# Autodesk Inventor assembly: Template A-I
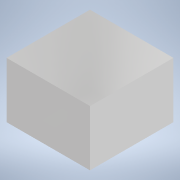
[picture p0: Inventor's stored thumbnail of the model, 180x180]
Saved by Autodesk Inventor 2022 (Build 260153000, 153)
## iProperties
Created: 2022-03-02
Part Number: Template A-I
Document SubType Name: Assembly
Designer: Nathan Griffith
Author: Nathan Griffith
## Documents named in this file (12)
- C:\Users\Nathan Griffith\Documents\Inventor\Eric's Keyboard\Template A-I.iam
- C:\Users\Nathan Griffith\Documents\Inventor\Eric's Keyboard\Block.ipt
- C:\Users\Nathan Griffith\Documents\Inventor\Eric's Keyboard\Keycap a-z\KeycapA.ipt
- C:\Users\Nathan Griffith\Documents\Inventor\Eric's Keyboard\Keycap a-z\KeycapB.ipt
- C:\Users\Nathan Griffith\Documents\Inventor\Eric's Keyboard\Keycap a-z\KeycapC.ipt
- C:\Users\Nathan Griffith\Documents\Inventor\Eric's Keyboard\Keycap a-z\KeycapD.ipt
- C:\Users\Nathan Griffith\Documents\Inventor\Eric's Keyboard\Keycap a-z\KeycapE.ipt
- C:\Users\Nathan Griffith\Documents\Inventor\Eric's Keyboard\Keycap a-z\KeycapF.ipt
- C:\Users\Nathan Griffith\Documents\Inventor\Eric's Keyboard\Keycap a-z\KeycapG.ipt
- C:\Users\Nathan Griffith\Documents\Inventor\Eric's Keyboard\Keycap a-z\KeycapH.ipt
- C:\Users\Nathan Griffith\Documents\Inventor\Eric's Keyboard\Keycap a-z\KeycapI.ipt
- C:\Users\Nathan Griffith\Documents\Inventor\Eric's Keyboard\Holder.iam
## Components (11 placed, 11 different names)
1. Block:1 — Mate:1, Mate:2, Mate:3, Mate:4, Mate:5, Mate:6, Mate:7, Mate:8, Mate:9, Mate:10, Mate:11, Mate:12, Mate:13, Mate:14, Mate:15, Mate:16, Mate:17, Mate:18
2. KeycapA:1 — Mate:1, Mate:2
3. KeycapB:1 — Mate:3, Mate:4
4. KeycapC:1 — Mate:5, Mate:6
5. KeycapD:1 — Mate:7, Mate:8
6. KeycapE:1 — Mate:9, Mate:10
7. KeycapF:1 — Mate:11, Mate:12
8. KeycapG:1 — Mate:13, Mate:14
9. KeycapH:1 — Mate:15, Mate:16
10. KeycapI:1 — Mate:17, Mate:18
11. Holder:1 [sub-assembly]
## Relationships (18: Mate 18)
- Mate:1: Block:1 ↔ KeycapA:1
- Mate:2: Block:1 ↔ KeycapA:1
- Mate:3: Block:1 ↔ KeycapB:1
- Mate:4: Block:1 ↔ KeycapB:1
- Mate:5: Block:1 ↔ KeycapC:1
- Mate:6: Block:1 ↔ KeycapC:1
- Mate:7: Block:1 ↔ KeycapD:1
- Mate:8: Block:1 ↔ KeycapD:1
- Mate:9: Block:1 ↔ KeycapE:1
- Mate:10: Block:1 ↔ KeycapE:1
- Mate:11: Block:1 ↔ KeycapF:1
- Mate:12: Block:1 ↔ KeycapF:1
- Mate:13: Block:1 ↔ KeycapG:1
- Mate:14: Block:1 ↔ KeycapG:1
- Mate:15: Block:1 ↔ KeycapH:1
- Mate:16: Block:1 ↔ KeycapH:1
- Mate:17: Block:1 ↔ KeycapI:1
- Mate:18: Block:1 ↔ KeycapI:1
